# Autodesk Inventor assembly: Assembly2
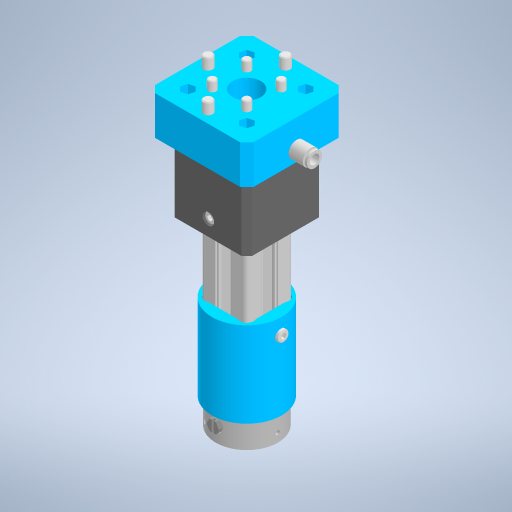
[picture p0: Inventor's stored thumbnail of the model, 512x512]
Saved by Autodesk Inventor 2023 (Build 270158000, 158)
## iProperties
Created: 2022-05-24
Part Number: Assembly2
Document SubType Name: Assembly
Designer: romanp
Author: romanp
## Documents named in this file (15)
- C:\Users\romanp\Desktop\SMC_End_Effector_Prototype\SMC_EE_XT661-4C-X427\Pack_and_Go\Assembly_SMC_EE.iam
- C:\Users\romanp\Desktop\SMC_End_Effector_Prototype\SMC_EE_XT661-4C-X427\Pack_and_Go\Part_Top_b_Blue.ipt
- C:\Users\romanp\Desktop\SMC_End_Effector_Prototype\SMC_EE_XT661-4C-X427\Pack_and_Go\ITEM30x30x100.ipt
- C:\Users\romanp\Desktop\SMC_End_Effector_Prototype\SMC_EE_XT661-4C-X427\Pack_and_Go\M4_nut.ipt
- C:\Users\romanp\Desktop\SMC_End_Effector_Prototype\SMC_EE_XT661-4C-X427\Pack_and_Go\Part_Bottom_Blue.ipt
- C:\Users\romanp\Desktop\SMC_End_Effector_Prototype\SMC_EE_XT661-4C-X427\Pack_and_Go\XT661-4C-X427.iam
- C:\Users\romanp\Desktop\SMC_End_Effector_Prototype\SMC_EE_XT661-4C-X427\Pack_and_Go\KQ2H06-M5N.ipt
- C:\Users\romanp\Desktop\SMC_End_Effector_Prototype\SMC_EE_XT661-4C-X427\Pack_and_Go\M4x20.ipt
- C:\Users\romanp\Desktop\SMC_End_Effector_Prototype\SMC_EE_XT661-4C-X427\Pack_and_Go\KQ2H06-00A.ipt
- C:\Users\romanp\Desktop\SMC_End_Effector_Prototype\SMC_EE_XT661-4C-X427\Pack_and_Go\M4x10.ipt
- C:\Users\romanp\Desktop\SMC_End_Effector_Prototype\SMC_EE_XT661-4C-X427\Pack_and_Go\Part_Middle_Black.ipt
- C:\Users\romanp\Desktop\SMC_End_Effector_Prototype\SMC_EE_XT661-4C-X427\Pack_and_Go\Part_Top_a_Blue.ipt
- C:\Users\romanp\Desktop\SMC_End_Effector_Prototype\SMC_EE_XT661-4C-X427\Pack_and_Go\hex_socket_cylindrical_head_M5x16.ipt
- C:\Users\romanp\Desktop\SMC_End_Effector_Prototype\SMC_EE_XT661-4C-X427\Pack_and_Go\hex_socket_cylindrical_head_M4x30.ipt
- C:\Users\romanp\Desktop\SMC_End_Effector_Prototype\SMC_EE_XT661-4C-X427\Pack_and_Go\hex_socket_cylindrical_head_M6x16.ipt
## Components (31 placed, 14 different names)
1. ITEM30x30x100:4 — Insert:70
2. KQ2H06-00A:1
3. Part_Bottom_Blue — Insert:57, Insert:58, Insert:60, Insert:61, Insert:62, Insert:63, Insert:64, Insert:65
4. M4x10:7 — Insert:64
5. XT661-4C-X427:3 [sub-assembly] — Insert:57, Insert:58, Insert:59
6. KQ2H06-M5N:3 — Insert:59
7. M4x20:7 — Insert:60
8. M4x20:8 — Insert:63
9. M4x20:9 — Insert:62
10. M4x20:10 — Insert:61
11. M4x10:8 — Insert:65
12. Part_Middle_Black:3 — Insert:70, Insert:71, Insert:73, Insert:74, Insert:79, Insert:80, Insert:81, Insert:82
13. Part_Top_a_Blue:1 — Insert:72, Insert:75, Insert:76, Insert:77, Insert:78, Insert:83, Insert:84, Insert:85, Insert:86, Insert:87, Insert:88, Insert:89
14. Part_Top_b_Blue:5 — Insert:71, Insert:72
15. M4x10:9 — Insert:73
16. M4x10:10 — Insert:74
17. M5x16:3 — Insert:75
18. M5x16:4 — Insert:76
19. M5x16:5 — Insert:78
20. M5x16:6 — Insert:77
21. M4x30:1 — Insert:80
22. M4x30:2 — Insert:81
23. M4x30:3 — Insert:82
24. M4x30:4 — Insert:79
25. M4_nut:7 — Insert:84
26. M4_nut:8 — Insert:86
27. M4_nut:9 — Insert:85
28. M4_nut:10 — Insert:83
29. M6x16:2 — Insert:89
30. M6x16:3 — Insert:88
31. M6x16:4 — Insert:87
## Relationships (29: Insert 29)
- Insert:57: Part_Bottom_Blue ↔ XT661-4C-X427:3
- Insert:58: Part_Bottom_Blue ↔ XT661-4C-X427:3
- Insert:59: XT661-4C-X427:3 ↔ KQ2H06-M5N:3
- Insert:60: Part_Bottom_Blue ↔ M4x20:7
- Insert:61: Part_Bottom_Blue ↔ M4x20:10
- Insert:62: Part_Bottom_Blue ↔ M4x20:9
- Insert:63: Part_Bottom_Blue ↔ M4x20:8
- Insert:64: Part_Bottom_Blue ↔ M4x10:7
- Insert:65: Part_Bottom_Blue ↔ M4x10:8
- Insert:70: ITEM30x30x100:4 ↔ Part_Middle_Black:3
- Insert:71: Part_Middle_Black:3 ↔ Part_Top_b_Blue:5
- Insert:72: Part_Top_a_Blue:1 ↔ Part_Top_b_Blue:5
- Insert:73: Part_Middle_Black:3 ↔ M4x10:9
- Insert:74: Part_Middle_Black:3 ↔ M4x10:10
- Insert:75: Part_Top_a_Blue:1 ↔ M5x16:3
- Insert:76: Part_Top_a_Blue:1 ↔ M5x16:4
- Insert:77: Part_Top_a_Blue:1 ↔ M5x16:6
- Insert:78: Part_Top_a_Blue:1 ↔ M5x16:5
- Insert:79: Part_Middle_Black:3 ↔ M4x30:4
- Insert:80: Part_Middle_Black:3 ↔ M4x30:1
- Insert:81: Part_Middle_Black:3 ↔ M4x30:2
- Insert:82: Part_Middle_Black:3 ↔ M4x30:3
- Insert:83: Part_Top_a_Blue:1 ↔ M4_nut:10
- Insert:84: Part_Top_a_Blue:1 ↔ M4_nut:7
- Insert:85: Part_Top_a_Blue:1 ↔ M4_nut:9
- Insert:86: Part_Top_a_Blue:1 ↔ M4_nut:8
- Insert:87: Part_Top_a_Blue:1 ↔ M6x16:4
- Insert:88: Part_Top_a_Blue:1 ↔ M6x16:3
- Insert:89: Part_Top_a_Blue:1 ↔ M6x16:2
